# Autodesk Inventor assembly: gear60
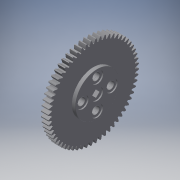
[picture p0: Inventor's stored thumbnail of the model, 180x180]
Saved by Autodesk Inventor 2019 (Build 230136000, 136)
## iProperties
Created: 2019-01-24
Part Number: gear60
Document SubType Name: Assembly
Designer: Varga Daniel
Author: Varga Daniel
## Documents named in this file (3)
- C:\!_Dani\!_cloud\OneDrive\!_munka\Revolution\RevvyDemoKit\Structural parts\Demo parts\Gears\gear60.iam
- C:\!_Dani\!_cloud\OneDrive\!_munka\Revolution\RevvyDemoKit\Structural parts\Demo parts\Gears\gear60.ipt
- C:\!_Dani\!_cloud\OneDrive\!_munka\Revolution\RevvyDemoKit\Structural parts\Demo parts\Gears\gear_collar.ipt
## Components (3 placed, 2 different names)
1. gear_collar:1 — Mate:6, Mate:7, Mate:8
2. gear60:1 — Mate:8, Mate:10
3. gear_collar:2 — Mate:6, Mate:7, Mate:10
## Relationships (4: Mate 4)
- Mate:6: gear_collar:1 ↔ gear_collar:2
- Mate:7: gear_collar:1 ↔ gear_collar:2
- Mate:8: gear_collar:1 ↔ gear60:1
- Mate:10: gear60:1 ↔ gear_collar:2
